# Autodesk Inventor assembly: Assembled box
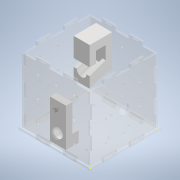
[picture p0: Inventor's stored thumbnail of the model, 180x180]
Saved by Autodesk Inventor 2021 (Build 250183000, 183)
## iProperties
Created: 2020-02-27
Part Number: Assembled box
Document SubType Name: Assembly
Designer: jstr255
Author: jstr255
## Documents named in this file (10)
- C:\Users\Jawal\Documents\UNI\PART III\Semester 1\MECHENG 334\Project A\CAD Files\Assemblies\Project_Cad_Files_export\Assemblies\Assembled box.iam
- C:\Users\Jawal\Documents\UNI\PART III\Semester 1\MECHENG 334\Project A\CAD Files\Box\Box base.ipt
- C:\Users\Jawal\Documents\UNI\PART III\Semester 1\MECHENG 334\Project A\CAD Files\Box\Box side 1.ipt
- C:\Users\Jawal\Documents\UNI\PART III\Semester 1\MECHENG 334\Project A\CAD Files\Box\Box side 2.ipt
- C:\Users\Jawal\Documents\UNI\PART III\Semester 1\MECHENG 334\Project A\CAD Files\Box\Box side 3.ipt
- C:\Users\Jawal\Documents\UNI\PART III\Semester 1\MECHENG 334\Project A\CAD Files\Box\Box side 4.ipt
- C:\Users\Jawal\Documents\UNI\PART III\Semester 1\MECHENG 334\Project A\CAD Files\Box\Box top.ipt
- C:\Users\Jawal\Documents\UNI\PART III\Semester 1\MECHENG 334\Project A\CAD Files\Ramp\Project_Cad_Files_export (2)\ramp\top_part.ipt
- C:\Users\Jawal\Documents\Inventor\Content Center Files\R2021\en-US\PN-86 M-82153\PN-86_M-82153 - M3 - 0.5.ipt
- C:\Users\Jawal\Documents\UNI\PART III\Semester 1\MECHENG 334\Project A\CAD Files\Ramp\Project_Cad_Files_export (2)\ramp\bottom_part.ipt
## Components (10 placed, 9 different names)
1. Box base:1 — Mate:1, Mate:2, Mate:3, Mate:4, Mate:5, Mate:6, Mate:7, Mate:8, Mate:9, Mate:10
2. Box side 1:1 — Mate:1, Mate:2, Mate:3, Flush:1, Mate:14
3. Box side 2:1 — Mate:4, Mate:5, Mate:6, Mate:13, Rigid:4, Rigid:5
4. Box side 3:1 — Mate:7, Mate:8, Mate:9, Mate:11
5. Box side 4:1 — Mate:10, Mate:11, Flush:1, Mate:12, Rigid:2, Rigid:3
6. Box top:1 — Mate:12, Mate:13, Mate:14
7. top_part:1 — Rigid:2
8. PN-86/M-82153 M3:1 — Rigid:3
9. bottom_part:1 — Rigid:4
10. PN-86/M-82153 M3:2 — Rigid:5
## Relationships (19: Mate 14, WeldJoint 4, Flush 1)
- Mate:1: Box base:1 ↔ Box side 1:1
- Mate:2: Box base:1 ↔ Box side 1:1
- Mate:3: Box base:1 ↔ Box side 1:1
- Mate:4: Box base:1 ↔ Box side 2:1
- Mate:5: Box base:1 ↔ Box side 2:1
- Mate:6: Box base:1 ↔ Box side 2:1
- Mate:7: Box base:1 ↔ Box side 3:1
- Mate:8: Box base:1 ↔ Box side 3:1
- Mate:9: Box base:1 ↔ Box side 3:1
- Mate:10: Box base:1 ↔ Box side 4:1
- Mate:11: Box side 3:1 ↔ Box side 4:1
- Flush:1: Box side 1:1 ↔ Box side 4:1
- Mate:12: Box side 4:1 ↔ Box top:1
- Mate:13: Box side 2:1 ↔ Box top:1
- Mate:14: Box side 1:1 ↔ Box top:1
- Rigid:2 [WeldJoint]: Box side 4:1 ↔ top_part:1
- Rigid:3 [WeldJoint]: Box side 4:1 ↔ PN-86/M-82153 M3:1
- Rigid:4 [WeldJoint]: Box side 2:1 ↔ bottom_part:1
- Rigid:5 [WeldJoint]: Box side 2:1 ↔ PN-86/M-82153 M3:2
